# Autodesk Inventor assembly: frame assembly
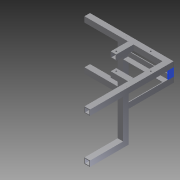
[picture p0: Inventor's stored thumbnail of the model, 180x180]
Saved by Autodesk Inventor 2012 (Build 160160000, 160)
## iProperties
Created: 2012-08-14
Part Number: frame assembly
Document SubType Name: Assembly
Designer: Bryce
Author: Bryce
## Documents named in this file (7)
- C:\Users\Bryce\Dropbox\Inventor Design Project Files\Independent Swerves\Inventor 2012\frame assembly.iam
- C:\Users\Bryce\Dropbox\Inventor Design Project Files\Independent Swerves\Inventor 2012\L frame.ipt
- C:\Users\Bryce\Dropbox\Inventor Design Project Files\Independent Swerves\Inventor 2012\Tube frame.ipt
- C:\Users\Bryce\Dropbox\Inventor Design Project Files\Independent Swerves\Inventor 2012\backwards L frame.ipt
- C:\Users\Bryce\Dropbox\Inventor Design Project Files\Independent Swerves\Inventor 2012\edge frame tube.ipt
- C:\Users\Bryce\Dropbox\Inventor Design Project Files\Independent Swerves\Inventor 2012\edge frame short.ipt
- C:\Users\Bryce\Dropbox\Inventor Design Project Files\Independent Swerves\Inventor 2012\L frame short.ipt
## Components (13 placed, 6 different names)
1. L frame:1 — Mate:1, Flush:1, Mate:2, Mate:3, Mate:4, Mate:37, Flush:14
2. Tube frame:1 — Mate:1, Flush:1, Mate:8, Mate:9, Mate:10
3. backwards L frame:1 — Mate:2, Mate:3, Mate:4, Mate:5, Mate:6, Mate:34, Flush:13
4. Tube frame:2 — Mate:5, Mate:6, Mate:11, Mate:12, Mate:13
5. Tube frame:3 — Mate:11, Mate:12, Mate:13, Mate:14, Mate:15, Mate:16, Mate:25
6. Tube frame:4 — Mate:8, Mate:9, Mate:10, Mate:17, Mate:18, Mate:19, Mate:26
7. Tube frame:5 — Mate:14, Mate:15, Mate:16, Flush:10
8. Tube frame:6 — Mate:17, Mate:18, Mate:19, Flush:7
9. edge frame tube:1 — Mate:23, Flush:6, Mate:24, Mate:25, Flush:10, Flush:11, Mate:35
10. edge frame tube:2 — Mate:23, Flush:6, Mate:24, Mate:26, Flush:7, Mate:34, Mate:36, Flush:12
11. edge frame short:1 — Mate:32, Mate:33, Flush:9, Flush:11, Mate:35
12. edge frame short:2 — Mate:32, Mate:33, Flush:9, Mate:36, Flush:12
13. L frame short:1 — Mate:37, Flush:13, Flush:14
## Relationships (37: Mate 28, Flush 9)
- Mate:1: L frame:1 ↔ Tube frame:1
- Flush:1: L frame:1 ↔ Tube frame:1
- Mate:2: L frame:1 ↔ backwards L frame:1
- Mate:3: L frame:1 ↔ backwards L frame:1
- Mate:4: L frame:1 ↔ backwards L frame:1
- Mate:5: backwards L frame:1 ↔ Tube frame:2
- Mate:6: backwards L frame:1 ↔ Tube frame:2
- Mate:8: Tube frame:1 ↔ Tube frame:4
- Mate:9: Tube frame:1 ↔ Tube frame:4
- Mate:10: Tube frame:1 ↔ Tube frame:4
- Mate:11: Tube frame:2 ↔ Tube frame:3
- Mate:12: Tube frame:2 ↔ Tube frame:3
- Mate:13: Tube frame:2 ↔ Tube frame:3
- Mate:14: Tube frame:3 ↔ Tube frame:5
- Mate:15: Tube frame:3 ↔ Tube frame:5
- Mate:16: Tube frame:3 ↔ Tube frame:5
- Mate:17: Tube frame:4 ↔ Tube frame:6
- Mate:18: Tube frame:4 ↔ Tube frame:6
- Mate:19: Tube frame:4 ↔ Tube frame:6
- Mate:23: edge frame tube:1 ↔ edge frame tube:2
- Flush:6: edge frame tube:1 ↔ edge frame tube:2
- Mate:24: edge frame tube:1 ↔ edge frame tube:2
- Mate:25: Tube frame:3 ↔ edge frame tube:1
- Mate:26: Tube frame:4 ↔ edge frame tube:2
- Flush:7: Tube frame:6 ↔ edge frame tube:2
- Mate:32: edge frame short:1 ↔ edge frame short:2
- Mate:33: edge frame short:1 ↔ edge frame short:2
- Flush:9: edge frame short:1 ↔ edge frame short:2
- Flush:10: Tube frame:5 ↔ edge frame tube:1
- Flush:11: edge frame tube:1 ↔ edge frame short:1
- Mate:34 (57.15 mm): backwards L frame:1 ↔ edge frame tube:2
- Mate:35: edge frame tube:1 ↔ edge frame short:1
- Mate:36: edge frame tube:2 ↔ edge frame short:2
- Flush:12: edge frame tube:2 ↔ edge frame short:2
- Mate:37: L frame:1 ↔ L frame short:1
- Flush:13: backwards L frame:1 ↔ L frame short:1
- Flush:14: L frame:1 ↔ L frame short:1
